# Autodesk Inventor assembly: RCPlaneAssembly
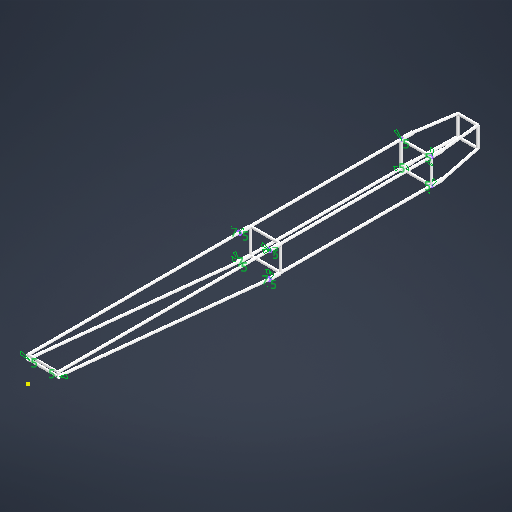
[picture p0: Inventor's stored thumbnail of the model, 512x512]
Saved by Autodesk Inventor 2026.1 (Build 301233000, 233)
## iProperties
Created: 2026-02-24
Part Number: RCPlaneAssembly
Document SubType Name: Assembly
Designer: morri
Mass: 90.2908 g
Surface Area: 689.687 cm^2
Volume: 82.0826 cm^3
Density: 1.1 g/cm^3
Author: morri
## Documents named in this file (4)
- C:\Users\morri\Documents\ENGR 2999 (Capstone)\RCPlaneAssembly.iam
- C:\Users\morri\Documents\ENGR 2999 (Capstone)\RCPlaneSkeletonMiddle1.ipt
- C:\Users\morri\Documents\ENGR 2999 (Capstone)\RCPlaneSkeletonTail1.ipt
- C:\Users\morri\Documents\ENGR 2999 (Capstone)\RCPlaneSkeletonFront1.ipt
## Components (3 placed, 3 different names)
1. RCPlaneSkeletonMiddle1:1 — Insert:2, Insert:3
2. RCPlaneSkeletonTail1:1 — Insert:3
3. RCPlaneSkeletonFront1:1 — Insert:2
## Relationships (2: Insert 2)
- Insert:2: RCPlaneSkeletonMiddle1:1 ↔ RCPlaneSkeletonFront1:1
- Insert:3: RCPlaneSkeletonMiddle1:1 ↔ RCPlaneSkeletonTail1:1
